# Autodesk Inventor assembly: vertPod
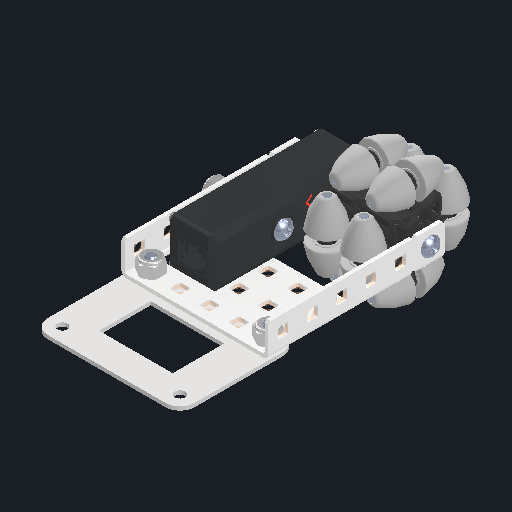
[picture p0: Inventor's stored thumbnail of the model, 512x512]
Saved by Autodesk Inventor 2026.1 (Build 301233000, 233)
## iProperties
Created: 2025-08-09
Part Number: vertPod
Document SubType Name: Assembly
Designer: roejo
Author: roejo
## Documents named in this file (18)
- C:\3284b-cad-2025\Robots\Highlander\SubAssemblies\vertPod.iam
- C:\3284b-cad-2025\Robots\Highlander\Poly\leafspringplate.ipt
- C:\3284b-cad-2025\Library\VEX-CAD-Inventor-1.4.2\Electronics\Sensors\V5 Rotation Sensor.ipt
- C:\3284b-cad-2025\Library\VEX-CAD-Inventor-1.4.2\Structure\Hardware\Nut Keps.ipt
- C:\Users\roejo\OneDrive\Documents\3284b-cad-2025\Library\VEX-CAD-Inventor-1.4.2\Motion\Spacers\Washer Teflon.ipt
- C:\3284b-cad-2025\Library\VEX-CAD-Inventor-1.4.2\Motion\Wheels\Omni Wheel\2 Omni AS, No Insert.ipt
- C:\3284b-cad-2025\Library\VEX-CAD-Inventor-1.4.2\Structure\Hardware\Nut Nylon\Nut Nylon - Black.ipt
- C:\Users\roejo\OneDrive\Documents\3284b-cad-2025\Library\VEX-CAD-Inventor-1.4.2\Structure\Hardware\Nut Nylon.ipt
- C:\3284b-cad-2025\Library\VEX-CAD-Inventor-1.4.2\Structure\Hardware\alu_nylock.ipt
- C:\Users\roejo\OneDrive\Documents\3284b-cad-2025\Library\VEX-CAD-Inventor-1.4.2\Structure\Hardware\Screw Steel - Star.ipt
- C:\3284b-cad-2025\Library\VEX-CAD-Inventor-1.4.2\Structure\Hardware\Screw Steel - Star\SScrew Star Smooth .500.ipt
- C:\3284b-cad-2025\Library\VEX-CAD-Inventor-1.4.2\Structure\Hardware\Screw Steel - Star\SScrew Star Smooth 1.500.ipt
- C:\Users\roejo\OneDrive\Documents\3284b-cad-2025\Library\VEX-CAD-Inventor-1.4.2\Motion\Spacers\Spacer Nylon .375 OD.ipt
- C:\3284b-cad-2025\Library\VEX-CAD-Inventor-1.4.2\Motion\Spacers\Spacer Nylon .375 OD\NSpacer .375 OD x .125.ipt
- C:\3284b-cad-2025\Library\VEX-CAD-Inventor-1.4.2\Structure\Hardware\Screw Steel - Star\SScrew Star Smooth 1.250.ipt
- C:\3284b-cad-2025\Robots\Highlander\Poly\leaf.ipt
- C:\3284b-cad-2025\Library\VEX-CAD-Inventor-1.4.2\Structure\Hardware\Screw Steel - Star\SScrew Star Smooth .375.ipt
- C:\3284b-cad-2025\Library\VEX-CAD-Inventor-1.4.2\Motion\Spacers\Washer Teflon\TWasher .375 OD x .03125.ipt
## Components (18 placed, 13 different names)
1. leafspringplate:1 — Insert:3, Insert:8, Insert:12, Insert:13, Insert:14, Insert:18, Insert:19, Insert:22, Insert:23
2. V5 Rotation Sensor:1 — Insert:7, Insert:17, Insert:25
3. Nut Keps:1 — Insert:3
4. Nut Nylon - Black:1 — Insert:7, Insert:8
5. alu_nylock:1 — Insert:12
6. SScrew Star Smooth .500:1 — Insert:13
7. SScrew Star Smooth 1.500:2 — Insert:14
8. SScrew Star Smooth 1.250:3 — Insert:17
9. leaf:1 — Insert:18, Insert:19, Insert:20, Insert:21
10. SScrew Star Smooth .375:4 — Insert:21
11. SScrew Star Smooth .375:5 — Insert:20
12. alu_nylock:2 — Insert:23
13. alu_nylock:3 — Insert:22
14. 2 Omni AS, No Insert:3 — Insert:28
15. 2 Omni AS, No Insert:4 — Insert:27
16. NSpacer .375 OD x .125:1 — Insert:25, Insert:26
17. TWasher .375 OD x .03125:1 — Insert:26, Insert:27
18. TWasher .375 OD x .03125:2 — Insert:28
## Relationships (18: Insert 18)
- Insert:3: leafspringplate:1 ↔ Nut Keps:1
- Insert:7: V5 Rotation Sensor:1 ↔ Nut Nylon - Black:1
- Insert:8: leafspringplate:1 ↔ Nut Nylon - Black:1
- Insert:12: leafspringplate:1 ↔ alu_nylock:1
- Insert:13: leafspringplate:1 ↔ SScrew Star Smooth .500:1
- Insert:14: leafspringplate:1 ↔ SScrew Star Smooth 1.500:2
- Insert:17: V5 Rotation Sensor:1 ↔ SScrew Star Smooth 1.250:3
- Insert:18: leafspringplate:1 ↔ leaf:1
- Insert:19: leafspringplate:1 ↔ leaf:1
- Insert:20: leaf:1 ↔ SScrew Star Smooth .375:5
- Insert:21: leaf:1 ↔ SScrew Star Smooth .375:4
- Insert:22: leafspringplate:1 ↔ alu_nylock:3
- Insert:23: leafspringplate:1 ↔ alu_nylock:2
- [Insert]: 2 Omni AS, No Insert:3 ↔ 2 Omni AS, No Insert:4
- Insert:25: V5 Rotation Sensor:1 ↔ NSpacer .375 OD x .125:1
- Insert:26: NSpacer .375 OD x .125:1 ↔ TWasher .375 OD x .03125:1
- Insert:27: 2 Omni AS, No Insert:4 ↔ TWasher .375 OD x .03125:1
- Insert:28: 2 Omni AS, No Insert:3 ↔ TWasher .375 OD x .03125:2
## Named parameters: d35_d5 = 0 mm
